# Autodesk Inventor assembly: s-assy-link2-bearing
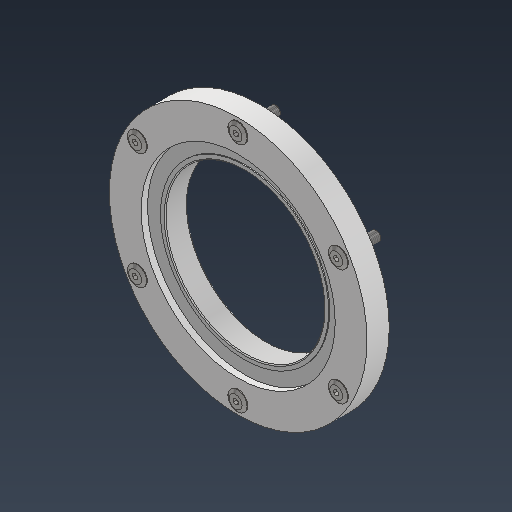
[picture p0: Inventor's stored thumbnail of the model, 512x512]
Saved by Autodesk Inventor 2021 (Build 250183000, 183)
## iProperties
Created: 2021-07-17
Part Number: s-assy-link2-bearing
Document SubType Name: Assembly
Designer: yuta0
Author: yuta0
## Documents named in this file (4)
- C:\Users\yuta0\Desktop\cat2021\catchrobo_arm\s-assy-link2-bearing.iam
- C:\Users\yuta0\Desktop\cat2021\catchrobo_arm\base2.ipt
- C:\Users\yuta0\Desktop\cat2021\catchrobo_arm\CBSTNR3-12.ipt
- C:\Users\yuta0\Desktop\cat2021\catchrobo_arm\B6810ZZ.ipt
## Components (8 placed, 3 different names)
1. base2:1 — メイト:3, メイト:4, メイト:5, メイト:6
2. B6810ZZ:1 — メイト:5, メイト:6
3. CBSTNR3-12:1 — メイト:3, メイト:4
4. CBSTNR3-12:2
5. CBSTNR3-12:3
6. CBSTNR3-12:4
7. CBSTNR3-12:5
8. CBSTNR3-12:6
## Component patterns: (6 elements, first: CBSTNR3-12:1)
## Relationships (4: Mate 4)
- メイト:3 [Mate]: base2:1 ↔ CBSTNR3-12:1
- メイト:4 [Mate]: base2:1 ↔ CBSTNR3-12:1
- メイト:5 [Mate]: base2:1 ↔ B6810ZZ:1
- メイト:6 [Mate]: base2:1 ↔ B6810ZZ:1
